# Autodesk Inventor assembly: birdeye_elbowUnit_actuator
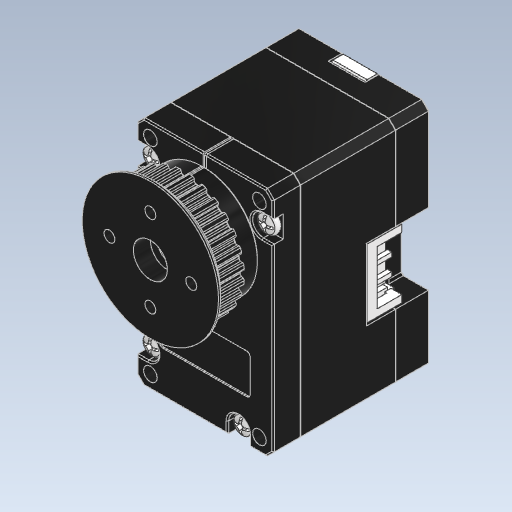
[picture p0: Inventor's stored thumbnail of the model, 512x512]
Saved by Autodesk Inventor 2024 (Build 280153000, 153)
## iProperties
Created: 2023-09-18
Part Number: birdeye_elbowUnit_actuator
Document SubType Name: Assembly
Designer: michi
Author: michi
## Documents named in this file (4)
- C:\Users\michi\OneDrive - Kyoto University\lab\6_SHINOBI\FUHGA4\Design_Mechanism\05_birdeye\birdeye_elbowUnit\birdeye_elbowUnit_actuator.iam
- C:\Users\michi\OneDrive - Kyoto University\lab\6_SHINOBI\FUHGA4\Design_Mechanism\00_devices\Dynamixel\X330\XL,XC-330.iam
- C:\Users\michi\OneDrive - Kyoto University\lab\6_SHINOBI\FUHGA4\Design_Mechanism\05_birdeye\birdeye_elbowUnit\brideye_elbowUnit_pully_active.ipt
- C:\Users\michi\OneDrive - Kyoto University\lab\6_SHINOBI\FUHGA4\Design_Mechanism\05_birdeye\birdeye_elbowUnit\_SPA-SUS-D1.6-6.ipt
## Components (6 placed, 3 different names)
1. XL,XC-330:1 [sub-assembly] — メイト:2, メイト:3, 回転:1
2. brideye_elbowUnit_pully_active:1 — メイト:4, 回転:1
3. _SPA-SUS-D1.6-6:1 — メイト:2, メイト:3, メイト:4
4. _SPA-SUS-D1.6-6:2
5. _SPA-SUS-D1.6-6:3
6. _SPA-SUS-D1.6-6:4
## Component patterns: (4 elements, first: _SPA-SUS-D1.6-6:1)
## Relationships (4: Mate 3, RevoluteJoint 1)
- メイト:2 [Mate]: XL,XC-330:1 ↔ _SPA-SUS-D1.6-6:1
- メイト:3 [Mate] (0.5 mm): XL,XC-330:1 ↔ _SPA-SUS-D1.6-6:1
- メイト:4 [Mate]: brideye_elbowUnit_pully_active:1 ↔ _SPA-SUS-D1.6-6:1
- 回転:1 [RevoluteJoint]: XL,XC-330:1 ↔ brideye_elbowUnit_pully_active:1
